# Autodesk Inventor assembly: SaponseEx
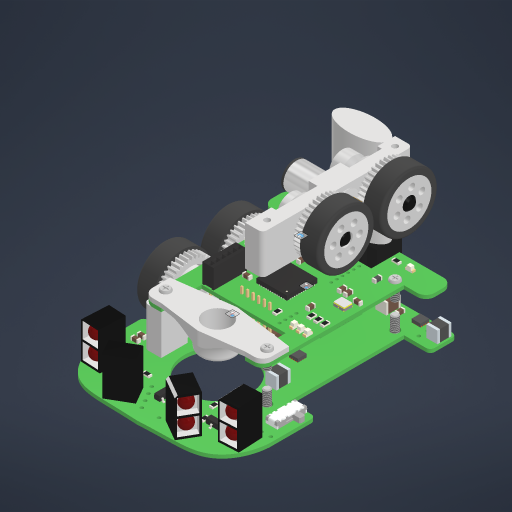
[picture p0: Inventor's stored thumbnail of the model, 512x512]
Saved by Autodesk Inventor 2023 (Build 270158000, 158)
## iProperties
Created: 2022-09-02
Part Number: SaponseEx
Document SubType Name: Assembly
Designer: neko2
Mass: 18.3356 g
Surface Area: 212.041 cm^2
Volume: 11.0257 cm^3
Density: 1.66299 g/cm^3
Author: neko2
## Documents named in this file (10)
- C:\Users\neko2\Desktop\SaponseEx\CAD\SaponseEx.iam
- C:\Users\neko2\Desktop\SaponseEx\CAD\足回り.iam
- C:\Users\neko2\Desktop\SaponseEx\CAD\PCB\SaponseEx_PCB.ipt
- C:\Users\neko2\Desktop\SaponseEx\CAD\Board_Parts\SNZS-M1_6-4.ipt
- C:\Users\neko2\Desktop\SaponseEx\CAD\PCB\Brains_PCB.ipt
- C:\Users\neko2\Desktop\SaponseEx\CAD\PCB\EncL_PCB.ipt
- C:\Users\neko2\Desktop\SaponseEx\CAD\PCB\EncR_PCB.ipt
- C:\Users\neko2\Desktop\SaponseEx\CAD\Board_Parts\Lipo.ipt
- C:\Users\neko2\Desktop\SaponseEx\CAD\吸引\FanMotorMount.ipt
- C:\Users\neko2\Desktop\SaponseEx\CAD\足回り_ミラー\足回り_MIR1.iam
## Components (16 placed, 9 different names)
1. SaponseEx_PCB:1 — フラッシュ:1, フラッシュ:2, メイト:1, リジッド:2, リジッド:3, メイト:2, リジッド:4, リジッド:5, メイト:10, メイト:11, メイト:12, メイト:19
2. 足回り:1 [sub-assembly] — 円柱状:1, 円柱状:2, メイト:2, 円柱状:5, メイト:14, 円柱状:7
3. Lipo:1 — メイト:10, メイト:11, メイト:12
4. FanMotorMount:1 — リジッド:8, リジッド:9, メイト:15
5. Brains_PCB:1 — リジッド:10, リジッド:11, メイト:14, メイト:15, メイト:17, メイト:18, フラッシュ:4, 円柱状:8
6. EncL_PCB:1 — メイト:16, メイト:17, フラッシュ:3, 対称度:1, フラッシュ:4
7. EncR_PCB:1 — メイト:16, メイト:18, フラッシュ:3, 対称度:1
8. 足回り_MIR1:1 [sub-assembly] — 円柱状:9, 円柱状:10, 円柱状:11
9. SNZS-M1_6-4:5 — 円柱状:5, リジッド:10
10. SNZS-M1_6-4:6 — リジッド:11, 円柱状:10
11. SNZS-M1_6-4:7 — リジッド:8, 円柱状:8, 円柱状:9
12. SNZS-M1_6-4:8 — リジッド:9, 円柱状:7
13. SNZS-M1_6-4:2 — リジッド:3, 円柱状:1
14. SNZS-M1_6-4:1 — リジッド:2, 円柱状:2
15. SNZS-M1_6-4:4 — リジッド:5
16. SNZS-M1_6-4:3 — リジッド:4, 円柱状:11
## Relationships (32: Mate 11, WeldJoint 8, CylindricalJoint 8, Flush 4, Symmetry 1)
- フラッシュ:1 [Flush]: SaponseEx_PCB:1
- フラッシュ:2 [Flush]: SaponseEx_PCB:1
- メイト:1 [Mate]: SaponseEx_PCB:1
- リジッド:2 [WeldJoint]: SaponseEx_PCB:1 ↔ SNZS-M1_6-4:1
- リジッド:3 [WeldJoint]: SaponseEx_PCB:1 ↔ SNZS-M1_6-4:2
- 円柱状:1 [CylindricalJoint]: 足回り:1 ↔ SNZS-M1_6-4:2
- 円柱状:2 [CylindricalJoint]: 足回り:1 ↔ SNZS-M1_6-4:1
- メイト:2 [Mate]: SaponseEx_PCB:1 ↔ 足回り:1
- リジッド:4 [WeldJoint]: SaponseEx_PCB:1 ↔ SNZS-M1_6-4:3
- リジッド:5 [WeldJoint]: SaponseEx_PCB:1 ↔ SNZS-M1_6-4:4
- 円柱状:5 [CylindricalJoint]: 足回り:1 ↔ SNZS-M1_6-4:5
- リジッド:8 [WeldJoint]: FanMotorMount:1 ↔ SNZS-M1_6-4:7
- リジッド:9 [WeldJoint]: FanMotorMount:1 ↔ SNZS-M1_6-4:8
- メイト:10 [Mate]: SaponseEx_PCB:1 ↔ Lipo:1
- メイト:11 [Mate]: SaponseEx_PCB:1 ↔ Lipo:1
- メイト:12 [Mate] (-0.1 mm): SaponseEx_PCB:1 ↔ Lipo:1
- リジッド:10 [WeldJoint]: Brains_PCB:1 ↔ SNZS-M1_6-4:5
- リジッド:11 [WeldJoint]: Brains_PCB:1 ↔ SNZS-M1_6-4:6
- メイト:14 [Mate]: 足回り:1 ↔ Brains_PCB:1
- メイト:15 [Mate]: FanMotorMount:1 ↔ Brains_PCB:1
- 円柱状:7 [CylindricalJoint]: 足回り:1 ↔ SNZS-M1_6-4:8
- メイト:16 [Mate] (7 mm): EncL_PCB:1 ↔ EncR_PCB:1
- メイト:17 [Mate]: Brains_PCB:1 ↔ EncL_PCB:1
- メイト:18 [Mate]: Brains_PCB:1 ↔ EncR_PCB:1
- フラッシュ:3 [Flush]: EncL_PCB:1 ↔ EncR_PCB:1
- 対称度:1 [Symmetry]: EncL_PCB:1 ↔ EncR_PCB:1
- メイト:19 [Mate]: SaponseEx_PCB:1
- フラッシュ:4 [Flush] (-0.2 mm): Brains_PCB:1 ↔ EncL_PCB:1
- 円柱状:8 [CylindricalJoint]: Brains_PCB:1 ↔ SNZS-M1_6-4:7
- 円柱状:9 [CylindricalJoint]: 足回り_MIR1:1 ↔ SNZS-M1_6-4:7
- 円柱状:10 [CylindricalJoint]: 足回り_MIR1:1 ↔ SNZS-M1_6-4:6
- 円柱状:11 [CylindricalJoint]: 足回り_MIR1:1 ↔ SNZS-M1_6-4:3
